# Autodesk Inventor assembly: enclosure_with_bracket
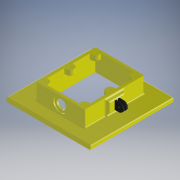
[picture p0: Inventor's stored thumbnail of the model, 180x180]
Saved by Autodesk Inventor 2018 (Build 220112000, 112)
## iProperties
Created: 2019-04-13
Part Number: enclosure_with_bracket
Document SubType Name: Assembly
Designer: ZEUSLAP
Author: ZEUSLAP
## Documents named in this file (3)
- C:\Users\ZEUSLAP\YandexDisk\Inventor\solar_harvester_145x145\enclosure\enclosure_with_bracket.iam
- C:\Users\ZEUSLAP\YandexDisk\Inventor\solar_harvester_145x145\enclosure\solar_panel_frame.ipt
- C:\Users\ZEUSLAP\YandexDisk\Inventor\solar_harvester_145x145\enclosure\camera_bracket\camera_bracket_male.ipt
## Components (2 placed, 2 different names)
1. solar_panel_frame:1 — Flush:1, Flush:2, Mate:1
2. camera_bracket_male:1 — Flush:1, Flush:2, Mate:1
## Relationships (3: Flush 2, Mate 1)
- Flush:1 (8 mm): solar_panel_frame:1 ↔ camera_bracket_male:1
- Flush:2 (50.5 mm): solar_panel_frame:1 ↔ camera_bracket_male:1
- Mate:1: solar_panel_frame:1 ↔ camera_bracket_male:1
